# Autodesk Inventor assembly: Ajedrez2
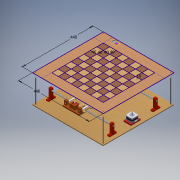
[picture p0: Inventor's stored thumbnail of the model, 180x180]
Saved by Autodesk Inventor 2019 (Build 230136000, 136)
## iProperties
Created: 2019-08-18
Part Number: Ajedrez2
Document SubType Name: Assembly
Designer: Bruno
Author: Bruno
## Documents named in this file (12)
- C:\Users\Bruno\Stuff\Ajedrez2\Ajedrez2.iam
- C:\Users\Bruno\Stuff\Ajedrez2\Floor.ipt
- C:\Users\Bruno\Stuff\Ajedrez2\XRodClamp.ipt
- C:\Users\Bruno\Stuff\Ajedrez2\XRod.ipt
- C:\Users\Bruno\Stuff\Ajedrez2\XMotor.iam
- C:\Users\Bruno\Stuff\Ajedrez2\XPulleySupport.iam
- C:\Users\Bruno\Stuff\Ajedrez2\XCart.iam
- C:\Users\Bruno\Stuff\Ajedrez2\YCart.iam
- C:\Users\Bruno\Stuff\Ajedrez2\Lid.iam
- C:\Users\Bruno\Stuff\Ajedrez\Inkjet Printer Prototype\Workspace\Wall.ipt
- C:\Users\Bruno\Stuff\Ajedrez\Inkjet Printer Prototype\Workspace\LidScrews.ipt
- C:\Users\Bruno\Stuff\Ajedrez2\Endstop mecânico - Chave fim de curso.ipt
## Components (19 placed, 11 different names)
1. Floor:1 — Flush:1, Flush:2, Rigid:7, Rigid:8, Rigid:9, Rigid:10, Rigid:11, Rigid:12, Flush:3, Flush:5, Flush:6, Rigid:13, Rigid:14, Rigid:15, Rigid:16
2. XRodClamp:1 — Rigid:5, Rigid:7
3. XRodClamp:2 — Rigid:10
4. XRodClamp:3 — Rigid:6, Rigid:8
5. XRodClamp:4 — Rigid:9
6. XRod:1 — Rigid:5, Cylindrical:2
7. XRod:2 — Rigid:6, Cylindrical:1
8. XMotor:1 [sub-assembly] — Rigid:11
9. XPulleySupport:1 [sub-assembly] — Rigid:12, Mate:1, Angle:1, Mate:2
10. XCart:1 [sub-assembly] — Cylindrical:1, Cylindrical:2, Cylindrical:3, Cylindrical:4, Mate:3, Rigid:17
11. YCart:1 [sub-assembly] — Cylindrical:3, Cylindrical:4
12. Lid:1 [sub-assembly] — Flush:1, Flush:2
13. Wall:1 — Flush:3, Flush:5
14. LidScrews:1 — Flush:6, Rigid:13
15. LidScrews:2 — Rigid:14
16. LidScrews:3 — Rigid:15
17. LidScrews:4 — Rigid:16
18. Endstop mecânico - Chave fim de curso:1 — Mate:1, Angle:1, Mate:2
19. Endstop mecânico - Chave fim de curso:2 — Mate:3, Rigid:17
## Relationships (26: WeldJoint 13, Flush 5, CylindricalJoint 4, Mate 3, Angle 1)
- Rigid:5 [WeldJoint]: XRodClamp:1 ↔ XRod:1
- Rigid:6 [WeldJoint]: XRodClamp:3 ↔ XRod:2
- Cylindrical:1: XRod:2 ↔ XCart:1
- Cylindrical:2: XRod:1 ↔ XCart:1
- Cylindrical:3: XCart:1 ↔ YCart:1
- Flush:1: Floor:1 ↔ Lid:1
- Flush:2: Floor:1 ↔ Lid:1
- Rigid:7 [WeldJoint]: Floor:1 ↔ XRodClamp:1
- Rigid:8 [WeldJoint]: Floor:1 ↔ XRodClamp:3
- Rigid:9 [WeldJoint]: Floor:1 ↔ XRodClamp:4
- Rigid:10 [WeldJoint]: Floor:1 ↔ XRodClamp:2
- Rigid:11 [WeldJoint]: Floor:1 ↔ XMotor:1
- Rigid:12 [WeldJoint]: Floor:1 ↔ XPulleySupport:1
- Flush:3: Floor:1 ↔ Wall:1
- Flush:5: Floor:1 ↔ Wall:1
- Cylindrical:4: XCart:1 ↔ YCart:1
- Flush:6: Floor:1 ↔ LidScrews:1
- Rigid:13 [WeldJoint]: Floor:1 ↔ LidScrews:1
- Rigid:14 [WeldJoint]: Floor:1 ↔ LidScrews:2
- Rigid:15 [WeldJoint]: Floor:1 ↔ LidScrews:3
- Rigid:16 [WeldJoint]: Floor:1 ↔ LidScrews:4
- Mate:1: XPulleySupport:1 ↔ Endstop mecânico - Chave fim de curso:1
- Angle:1 (0 deg): XPulleySupport:1 ↔ Endstop mecânico - Chave fim de curso:1
- Mate:2: XPulleySupport:1 ↔ Endstop mecânico - Chave fim de curso:1
- Mate:3: XCart:1 ↔ Endstop mecânico - Chave fim de curso:2
- Rigid:17 [WeldJoint]: XCart:1 ↔ Endstop mecânico - Chave fim de curso:2
